# Autodesk Inventor assembly: fullbodyAssembly
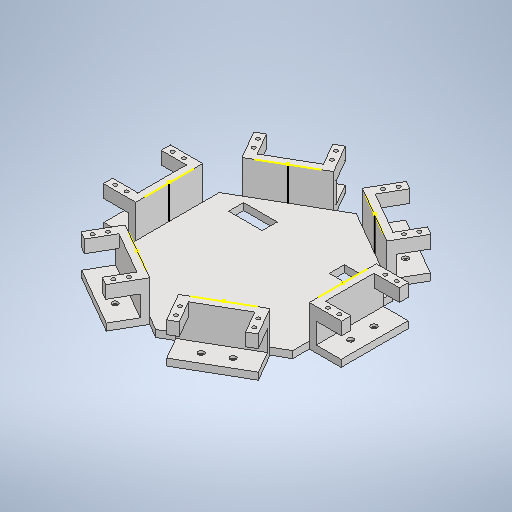
[picture p0: Inventor's stored thumbnail of the model, 512x512]
Saved by Autodesk Inventor 2025.1 (Build 291241020, 241B)
## iProperties
Created: 2025-03-08
Part Number: fullbodyAssembly
Document SubType Name: Assembly
Designer: omiye
Author: omiye
## Documents named in this file (3)
- C:\Projects\Arduino\hexapod\legModels\fullbodyAssembly.iam
- C:\Projects\Arduino\hexapod\legModels\baseBody.ipt
- C:\Projects\Arduino\hexapod\legModels\servoBody.ipt
## Components (7 placed, 2 different names)
1. baseBody:1 — Mate:1, Mate:2, Mate:3, Mate:4, Mate:5, Mate:6, Mate:7, Mate:8, Mate:9, Mate:10, Mate:11, Mate:12, Flush:1, Flush:2, Flush:3, Flush:4, Flush:5, Flush:6
2. servoBody:1 — Mate:1, Mate:2, Flush:2
3. servoBody:2 — Mate:3, Mate:4, Flush:1
4. servoBody:3 — Mate:5, Mate:6, Flush:6
5. servoBody:4 — Mate:11, Mate:12, Flush:3
6. servoBody:5 — Mate:7, Mate:8, Flush:5
7. servoBody:6 — Mate:9, Mate:10, Flush:4
## Relationships (18: Mate 12, Flush 6)
- Mate:1: baseBody:1 ↔ servoBody:1
- Mate:2: baseBody:1 ↔ servoBody:1
- Mate:3: baseBody:1 ↔ servoBody:2
- Mate:4: baseBody:1 ↔ servoBody:2
- Mate:5: baseBody:1 ↔ servoBody:3
- Mate:6: baseBody:1 ↔ servoBody:3
- Mate:7: baseBody:1 ↔ servoBody:5
- Mate:8: baseBody:1 ↔ servoBody:5
- Mate:9: baseBody:1 ↔ servoBody:6
- Mate:10: baseBody:1 ↔ servoBody:6
- Mate:11: baseBody:1 ↔ servoBody:4
- Mate:12: baseBody:1 ↔ servoBody:4
- Flush:1: baseBody:1 ↔ servoBody:2
- Flush:2: baseBody:1 ↔ servoBody:1
- Flush:3: baseBody:1 ↔ servoBody:4
- Flush:4: baseBody:1 ↔ servoBody:6
- Flush:5: baseBody:1 ↔ servoBody:5
- Flush:6: baseBody:1 ↔ servoBody:3
